# Autodesk Inventor assembly: Bot Assembly v3
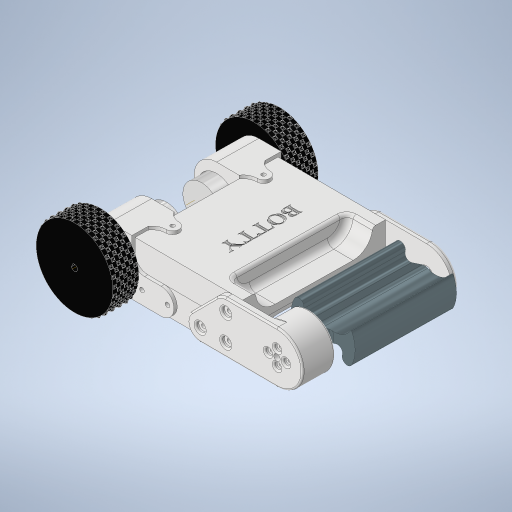
[picture p0: Inventor's stored thumbnail of the model, 512x512]
Saved by Autodesk Inventor 2024 (Build 280153000, 153)
## iProperties
Created: 2023-11-27
Part Number: Bot Assembly v3
Document SubType Name: Assembly
Designer: CJ110
Author: CJ110
## Documents named in this file (11)
- D:\GitHub\Vault-1\CAD\WCRL\Bot Assembly v3.iam
- D:\GitHub\Vault-1\CAD\WCRL\hub.ipt
- D:\GitHub\Vault-1\CAD\WCRL\Motor Mount left.ipt
- D:\GitHub\Vault-1\CAD\WCRL\Motor Mount right.ipt
- D:\GitHub\Vault-1\CAD\WCRL\DC 12V 200RPM.ipt
- D:\GitHub\Vault-1\CAD\WCRL\WHEEL_SPIKEY_smallspikes.ipt
- D:\GitHub\Vault-1\CAD\WCRL\Bearing Bracket.ipt
- D:\GitHub\Vault-1\CAD\WCRL\BLDC Bracket.ipt
- D:\GitHub\Vault-1\CAD\WCRL\drum2.ipt
- D:\GitHub\Vault-1\CAD\WCRL\Brushless 2622 2600KV.ipt
- D:\GitHub\Vault-1\CAD\WCRL\Top v2.ipt
## Components (12 placed, 10 different names)
1. hub:1 — Mate:1, Mate:2, Mate:3, Mate:4, Mate:5, Mate:6, Mate:19, Mate:22, Mate:27, Mate:28, Mate:29, Mate:30, Mate:31, Flush:1, Flush:2
2. Motor Mount left:1 — Mate:4, Mate:5, Mate:6, Mate:8, Mate:9, Mate:10
3. Motor Mount right:1 — Mate:1, Mate:2, Mate:3, Mate:7, Mate:11, Mate:12
4. DC 12V 200RPM:1 — Mate:7, Mate:11, Mate:12, Mate:13, Mate:15
5. DC 12V 200RPM:2 — Mate:8, Mate:9, Mate:10, Mate:14, Mate:16
6. WHEEL_SPIKEY_smallspikes:1 — Mate:13, Mate:15
7. WHEEL_SPIKEY_smallspikes:2 — Mate:14, Mate:16
8. Bearing Bracket:1 — Mate:19, Mate:23, Mate:29, Mate:30
9. BLDC Bracket:1 — Mate:22, Mate:24, Mate:26, Mate:27, Mate:28
10. drum2:1 — Mate:23, Mate:25
11. Brushless 2622 2600KV:1 — Mate:24, Mate:25, Mate:26
12. Top v2:1 — Mate:31, Flush:1, Flush:2
## Relationships (29: Mate 27, Flush 2)
- Mate:1: hub:1 ↔ Motor Mount right:1
- Mate:2: hub:1 ↔ Motor Mount right:1
- Mate:3: hub:1 ↔ Motor Mount right:1
- Mate:4: hub:1 ↔ Motor Mount left:1
- Mate:5: hub:1 ↔ Motor Mount left:1
- Mate:6: hub:1 ↔ Motor Mount left:1
- Mate:7: Motor Mount right:1 ↔ DC 12V 200RPM:1
- Mate:8: Motor Mount left:1 ↔ DC 12V 200RPM:2
- Mate:9: Motor Mount left:1 ↔ DC 12V 200RPM:2
- Mate:10: Motor Mount left:1 ↔ DC 12V 200RPM:2
- Mate:11: Motor Mount right:1 ↔ DC 12V 200RPM:1
- Mate:12: Motor Mount right:1 ↔ DC 12V 200RPM:1
- Mate:13: DC 12V 200RPM:1 ↔ WHEEL_SPIKEY_smallspikes:1
- Mate:14: DC 12V 200RPM:2 ↔ WHEEL_SPIKEY_smallspikes:2
- Mate:15: DC 12V 200RPM:1 ↔ WHEEL_SPIKEY_smallspikes:1
- Mate:16: DC 12V 200RPM:2 ↔ WHEEL_SPIKEY_smallspikes:2
- Mate:19: hub:1 ↔ Bearing Bracket:1
- Mate:22: hub:1 ↔ BLDC Bracket:1
- Mate:23: Bearing Bracket:1 ↔ drum2:1
- Mate:24: BLDC Bracket:1 ↔ Brushless 2622 2600KV:1
- Mate:25: drum2:1 ↔ Brushless 2622 2600KV:1
- Mate:26: BLDC Bracket:1 ↔ Brushless 2622 2600KV:1
- Mate:27: hub:1 ↔ BLDC Bracket:1
- Mate:28: hub:1 ↔ BLDC Bracket:1
- Mate:29: hub:1 ↔ Bearing Bracket:1
- Mate:30: hub:1 ↔ Bearing Bracket:1
- Mate:31: hub:1 ↔ Top v2:1
- Flush:1: hub:1 ↔ Top v2:1
- Flush:2: hub:1 ↔ Top v2:1
